# Autodesk Inventor assembly: 2018 Build Model
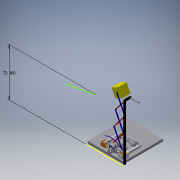
[picture p0: Inventor's stored thumbnail of the model, 180x180]
Saved by Autodesk Inventor 2018 (Build 220112000, 112)
## iProperties
Created: 2016-01-11
Part Number: 2018 Build Model
Document SubType Name: Assembly
Designer: Applegate
Author: Applegate
## Documents named in this file (11)
- C:\Users\Apple\Documents\Inventor\2018 PowerUp\2018 Build Model.iam
- C:\Users\Apple\Documents\Inventor\2018 PowerUp\2016_Files_2018_Mod\Sissor Lift\Long Bar.ipt
- C:\Users\Apple\Documents\Inventor\2018 PowerUp\2016_Files_2018_Mod\Sissor Lift\Gounded Clevis.ipt
- C:\Users\Apple\Documents\Inventor\2018 PowerUp\2016_Files_2018_Mod\Sissor Lift\Long Bar Offset center.ipt
- C:\Users\Apple\Documents\Inventor\2018 PowerUp\Ramp.ipt
- C:\Users\Apple\Documents\Inventor\2018 PowerUp\Vertical Rung.ipt
- C:\Users\Apple\Documents\Inventor\2018 PowerUp\Rung Support.ipt
- C:\Users\Apple\Documents\Inventor\2018 PowerUp\Rung Bar.ipt
- C:\Users\Apple\Documents\Inventor\2018 PowerUp\2016_Files_2018_Mod\Assembly\My Chassy.iam
- C:\Users\Apple\Documents\Inventor\2018 PowerUp\2016_Files_2018_Mod\Sissor Lift\PowerCube.ipt
- am-2951 AM14U2 Outside Sheet.ipt
## Components (13 placed, 9 different names)
1. Gounded Clevis:1 — Rotational:3, FrontSissorAnchor, Flush:13, Flush:14
2. Long Bar:1 — Rotational:3, Rotational:4, Rotational:6
3. Long Bar:2 — Rotational:5, Rotational:7, Rotational:10
4. Long Bar Offset center:1 — Rotational:4, Rotational:5, Rear Sissor Slide
5. Long Bar Offset center:2 — Rotational:6, Rotational:7, Rotational:8
6. Ramp:1 — Flush:1, Flush:4, Mate:4, Flush:5, Mate:10, Flush:11, Flush:12, Flush:16
7. Vertical Rung:1 — Flush:4, Mate:4, Flush:5, Flush:7, Mate:7, Flush:10
8. Rung Support:1 — Flush:7, Flush:9, Mate:6, Mate:7, Flush:10
9. Rung Bar:1 — Flush:9, Mate:6
10. Long Bar:3 — Rotational:8, Rotational:9, Angle:1
11. Long Bar Offset center:3 — Rotational:9, Rotational:10
12. My Chassy:1 [sub-assembly] — Mate:10, Flush:11, Flush:12, Flush:13, Flush:14, FrontSissorAnchor, Rear Sissor Slide, Flush:15
13. PowerCube:1 — Flush:16, Angle:1
## Relationships (27: Flush 12, RevoluteJoint 8, Mate 6, Angle 1)
- Rotational:3 [RevoluteJoint]: Gounded Clevis:1 ↔ Long Bar:1
- Rotational:4 [RevoluteJoint]: Long Bar:1 ↔ Long Bar Offset center:1
- Rotational:5 [RevoluteJoint]: Long Bar:2 ↔ Long Bar Offset center:1
- Rotational:6 [RevoluteJoint]: Long Bar:1 ↔ Long Bar Offset center:2
- Rotational:7 [RevoluteJoint]: Long Bar:2 ↔ Long Bar Offset center:2
- Flush:1: Ramp:1
- Flush:4: Ramp:1 ↔ Vertical Rung:1
- Mate:4: Ramp:1 ↔ Vertical Rung:1
- Flush:5: Ramp:1 ↔ Vertical Rung:1
- Flush:7: Vertical Rung:1 ↔ Rung Support:1
- Flush:9: Rung Support:1 ↔ Rung Bar:1
- Mate:6: Rung Support:1 ↔ Rung Bar:1
- Mate:7: Vertical Rung:1 ↔ Rung Support:1
- Flush:10: Vertical Rung:1 ↔ Rung Support:1
- Rotational:8 [RevoluteJoint]: Long Bar Offset center:2 ↔ Long Bar:3
- Rotational:9 [RevoluteJoint]: Long Bar:3 ↔ Long Bar Offset center:3
- Rotational:10 [RevoluteJoint]: Long Bar:2 ↔ Long Bar Offset center:3
- Mate:10 (63.5 mm): Ramp:1 ↔ My Chassy:1
- Flush:11 (76.2 mm): Ramp:1 ↔ My Chassy:1
- Flush:12 (76.2 mm): Ramp:1 ↔ My Chassy:1
- Flush:13 (76.2 mm): Gounded Clevis:1 ↔ My Chassy:1
- Flush:14 (21.6408 mm): Gounded Clevis:1 ↔ My Chassy:1
- FrontSissorAnchor [Mate] (101.6 mm): Gounded Clevis:1 ↔ My Chassy:1
- Rear Sissor Slide [Mate] (152.4 mm): Long Bar Offset center:1 ↔ My Chassy:1
- Flush:15 (127 mm): My Chassy:1
- Flush:16: Ramp:1 ↔ PowerCube:1
- Angle:1 (0 deg): Long Bar:3 ↔ PowerCube:1
